# Autodesk Inventor assembly: finish_assembly_1
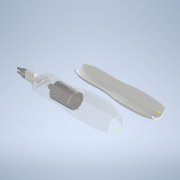
[picture p0: Inventor's stored thumbnail of the model, 180x180]
Saved by Autodesk Inventor 2020 (Build 240168000, 168)
## iProperties
Created: 2020-02-11
Part Number: finish_assembly_1
Document SubType Name: Assembly
Designer: metal
Author: metal
## Documents named in this file (10)
- C:\Polyimide_isolation_cleaner\finish_assembly_1.iam
- C:\Polyimide_isolation_cleaner\korob_3.ipt
- C:\Polyimide_isolation_cleaner\pielers2.ipt
- C:\Polyimide_isolation_cleaner\pielers.ipt
- C:\Polyimide_isolation_cleaner\R370-25120.ipt
- C:\Polyimide_isolation_cleaner\blade.ipt
- C:\Polyimide_isolation_cleaner\plastic_case_3.2_BACK.ipt
- C:\Polyimide_isolation_cleaner\excentrick_2.ipt
- C:\Polyimide_isolation_cleaner\направляющая.ipt
- C:\Polyimide_isolation_cleaner\plastic_case_3.2_TOP.ipt
## Components (11 placed, 9 different names)
1. korob_3:1 — Rigid:1, Slider:1
2. pielers2:1 — Rotational:1, Rigid:9
3. pielers:1 — Rigid:1, Rotational:1, Rigid:10
4. R370-25120:1 — Rotational:2, Mate:1, Mate:2, Mate:3
5. blade:1 — Rigid:10
6. blade:2 — Rigid:9
7. plastic_case_3.2_BACK:1 — Slider:1, Mate:1, Mate:2, Rigid:11, Rigid:12, Mate:3
8. excentrick_2:1 — Rotational:2
9. направляющая:1 — Rigid:11
10. направляющая:2 — Rigid:12
11. plastic_case_3.2_TOP:1
## Relationships (11: WeldJoint 5, Mate 3, RevoluteJoint 2, TranslationJoint 1)
- Rigid:1 [WeldJoint]: korob_3:1 ↔ pielers:1
- Rotational:1 [RevoluteJoint] (-0.4 mm): pielers2:1 ↔ pielers:1
- Rigid:9 [WeldJoint]: pielers2:1 ↔ blade:2
- Rigid:10 [WeldJoint]: pielers:1 ↔ blade:1
- Rotational:2 [RevoluteJoint]: R370-25120:1 ↔ excentrick_2:1
- Slider:1 [TranslationJoint]: korob_3:1 ↔ plastic_case_3.2_BACK:1
- Mate:1: R370-25120:1 ↔ plastic_case_3.2_BACK:1
- Mate:2: R370-25120:1 ↔ plastic_case_3.2_BACK:1
- Rigid:11 [WeldJoint]: plastic_case_3.2_BACK:1 ↔ направляющая:1
- Rigid:12 [WeldJoint]: plastic_case_3.2_BACK:1 ↔ направляющая:2
- Mate:3: R370-25120:1 ↔ plastic_case_3.2_BACK:1
